# Autodesk Inventor assembly: arm_holder
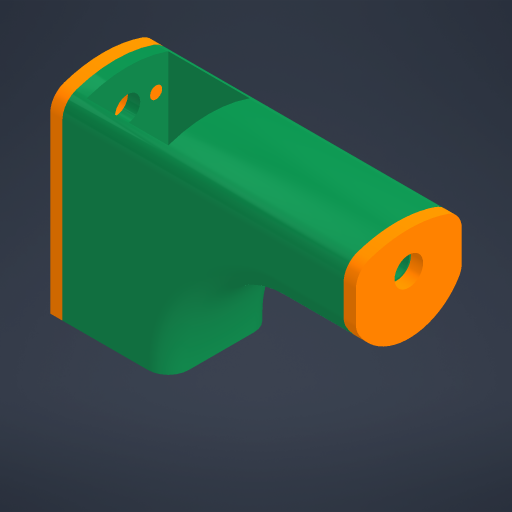
[picture p0: Inventor's stored thumbnail of the model, 512x512]
Saved by Autodesk Inventor 2024 (Build 280153000, 153)
## iProperties
Created: 2023-11-08
Part Number: arm_holder
Document SubType Name: Assembly
Designer: user
Author: user
## Documents named in this file (4)
- D:\Docs\Robot\3d_v2\machine_body\arm_assembly\arm_holder.iam
- D:\Docs\Robot\3d_v2\machine_body\arm_assembly\arm_holder.ipt
- D:\Docs\Robot\3d_v2\machine_body\arm_assembly\gasket\gasket_1.ipt
- D:\Docs\Robot\3d_v2\machine_body\arm_assembly\gasket\gasket_2.ipt
## Components (3 placed, 3 different names)
1. arm_holder:1 — Заподлицо:1, Заподлицо:2, Совмещение:1, Заподлицо:3, Заподлицо:4
2. gasket_1:1 — Заподлицо:3
3. gasket_2:1 — Заподлицо:4
## Relationships (5: Flush 4, Mate 1)
- Заподлицо:1 [Flush]: arm_holder:1
- Заподлицо:2 [Flush]: arm_holder:1
- Совмещение:1 [Mate]: arm_holder:1
- Заподлицо:3 [Flush]: arm_holder:1 ↔ gasket_1:1
- Заподлицо:4 [Flush]: arm_holder:1 ↔ gasket_2:1
